# Autodesk Inventor assembly: A_Aft
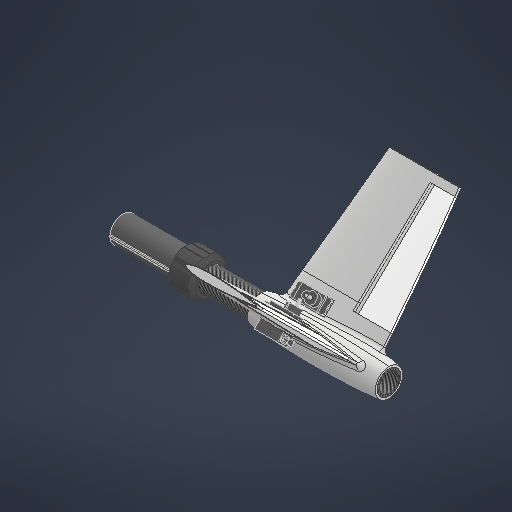
[picture p0: Inventor's stored thumbnail of the model, 512x512]
Saved by Autodesk Inventor 2026 (Build 300175000, 175)
## iProperties
Created: 2025-09-10
Part Number: A_Aft
Document SubType Name: Assembly
Designer: FAL
Author: FAL
## Documents named in this file (8)
- C:\Users\FAL\Projekte\Git\AIRBERT\CAD\Aft\A_Aft.iam
- C:\Users\FAL\Projekte\Git\AIRBERT\CAD\Aft\P_aft_V.ipt
- C:\Users\FAL\Projekte\Git\AIRBERT\CAD\Aft\P_aft_V_rudder.ipt
- C:\Users\FAL\Projekte\Git\AIRBERT\CAD\Aft\P_Carbon_Pipe_Back.ipt
- C:\Users\FAL\Projekte\Git\AIRBERT\CAD\Electronic\P_Servo_27x12.ipt
- C:\Users\FAL\Projekte\Git\AIRBERT\CAD\Aft\P_Aft_body_pipe_connector_inlet_movable.ipt
- C:\Users\FAL\Projekte\Git\AIRBERT\CAD\Aft\P_aft_body_pipe_connector_nut.ipt
- C:\Users\FAL\Projekte\Git\AIRBERT\CAD\Aft\mirror\P_aft_V_rudder_MIR1.ipt
## Components (8 placed, 7 different names)
1. P_aft_V:1 — Passend:12, Fluchtend:20, Fluchtend:21, Fluchtend:22, Fluchtend:23, Fluchtend:24, Passend:13, Passend:14, Passend:15, Passend:16, Passend:17, Passend:18
2. P_aft_V_rudder:1 — Fluchtend:22, Fluchtend:23, Fluchtend:24
3. P_Carbon_Pipe_Back:1 — Passend:11, Fluchtend:19, Passend:12, Fluchtend:21
4. P_Servo_27x12:1 — Passend:14, Passend:15, Passend:16
5. P_Servo_27x12:2 — Passend:13, Passend:17, Passend:18
6. P_Aft_body_pipe_connector_inlet_movable:1 — Fluchtend:16, Fluchtend:17, Fluchtend:18, Fluchtend:19
7. P_aft_body_pipe_connector_nut:1 — Fluchtend:13, Fluchtend:14, Fluchtend:15
8. P_aft_V_rudder_MIR1:1
## Relationships (20: Flush 12, Mate 8)
- Fluchtend:13 [Flush]: P_aft_body_pipe_connector_nut:1
- Fluchtend:14 [Flush]: P_aft_body_pipe_connector_nut:1
- Fluchtend:15 [Flush]: P_aft_body_pipe_connector_nut:1
- Passend:11 [Mate]: P_Carbon_Pipe_Back:1
- Fluchtend:16 [Flush]: P_Aft_body_pipe_connector_inlet_movable:1
- Fluchtend:17 [Flush]: P_Aft_body_pipe_connector_inlet_movable:1
- Fluchtend:18 [Flush]: P_Aft_body_pipe_connector_inlet_movable:1
- Fluchtend:19 [Flush]: P_Carbon_Pipe_Back:1 ↔ P_Aft_body_pipe_connector_inlet_movable:1
- Passend:12 [Mate]: P_aft_V:1 ↔ P_Carbon_Pipe_Back:1
- Fluchtend:20 [Flush]: P_aft_V:1
- Fluchtend:21 [Flush]: P_aft_V:1 ↔ P_Carbon_Pipe_Back:1
- Fluchtend:22 [Flush]: P_aft_V:1 ↔ P_aft_V_rudder:1
- Fluchtend:23 [Flush]: P_aft_V:1 ↔ P_aft_V_rudder:1
- Fluchtend:24 [Flush]: P_aft_V:1 ↔ P_aft_V_rudder:1
- Passend:13 [Mate]: P_aft_V:1 ↔ P_Servo_27x12:2
- Passend:14 [Mate]: P_aft_V:1 ↔ P_Servo_27x12:1
- Passend:15 [Mate]: P_aft_V:1 ↔ P_Servo_27x12:1
- Passend:16 [Mate]: P_aft_V:1 ↔ P_Servo_27x12:1
- Passend:17 [Mate]: P_aft_V:1 ↔ P_Servo_27x12:2
- Passend:18 [Mate]: P_aft_V:1 ↔ P_Servo_27x12:2
